# Autodesk Inventor assembly: Naped
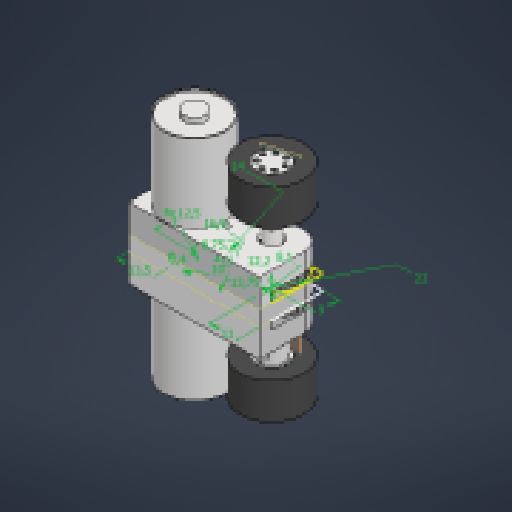
[picture p0: Inventor's stored thumbnail of the model, 512x512]
Saved by Autodesk Inventor 2023 (Build 270158000, 158)
## iProperties
Created: 2024-02-25
Part Number: Naped
Document SubType Name: Assembly
Designer: Michał
Author: Michał
## Documents named in this file (16)
- D:\Projekty\Roboilo\Ser\3D\3D\V2\Naped.iam
- D:\Projekty\Roboilo\Ser\3D\3D\V2\Naped\Przegroda.ipt
- D:\Projekty\Roboilo\Ser\3D\3D\V2\Naped\MocowaniePrzekladni.ipt
- D:\Projekty\Roboilo\Ser\3D\3D\PrzekladniaLewa\Design Accelerator\Przekładnie walcowe2.iam
- D:\Projekty\Roboilo\Ser\3D\3D\PrzekladniaLewa\Design Accelerator\Przekładnie walcowe3.iam
- D:\Projekty\Roboilo\Ser\3D\3D\PrzekladniaLewa\Design Accelerator\Przekładnie walcowe4.iam
- D:\Projekty\Roboilo\Ser\3D\3D\V2\Silnik.ipt
- D:\Projekty\Roboilo\Ser\3D\3D\V2\Naped\kolo.iam
- D:\Projekty\Roboilo\Ser\3D\3D\V2\Naped\Lozysko GFM-0608-06.ipt
- D:\Projekty\Roboilo\Ser\3D\3D\V2\Naped\MocowaniePrzekladni_MIR1.ipt
- D:\Projekty\Roboilo\Ser\3D\3D\V2\Silnik_MIR.ipt
- D:\Projekty\Roboilo\Ser\3D\3D\V2\Naped\kolo_MIR.iam
- D:\Projekty\Roboilo\Ser\3D\3D\PrzekladniaLewa\Design Accelerator\Przekładnie walcowe2_MIR.iam
- D:\Projekty\Roboilo\Ser\3D\3D\PrzekladniaLewa\Design Accelerator\Przekładnie walcowe3_MIR.iam
- D:\Projekty\Roboilo\Ser\3D\3D\PrzekladniaLewa\Design Accelerator\Przekładnie walcowe4_MIR.iam
- D:\Projekty\Roboilo\Ser\3D\3D\V2\Naped\Lozysko GFM-0608-06_MIR.ipt
## Components (15 placed, 13 different names)
1. Przegroda:1 — Flush:1, Flush:2, Mate:1, Mate:16, Flush:3, Flush:4
2. MocowaniePrzekladni:1 — Flush:1, Flush:2, Mate:1, Insert:1, Insert:2, Insert:3, Mate:3, Mate:4, Mate:5, Mate:6
3. Silnik:1 — Insert:1, Insert:2
4. kolo:1 [sub-assembly] — Mate:7, Mate:8
5. Przekładnie walcowe:1 [sub-assembly] — Insert:5, Mate:5, Mate:6
6. Przekładnie walcowe:2 [sub-assembly] — Insert:4, Insert:5, Mate:4
7. Przekładnie walcowe:3 [sub-assembly] — Insert:4, Mate:2, Mate:3, Mate:7, Mate:8
8. Lozysko GFM-0608-06:1 — Insert:3, Mate:2
9. MocowaniePrzekladni_MIR1:1 — Insert:6, Insert:7, Mate:9, Mate:10, Mate:11, Mate:14, Insert:10, Mate:16, Flush:3, Flush:4
10. Silnik_MIR:1 — Insert:6, Insert:7
11. kolo_MIR:1 [sub-assembly] — Mate:12, Mate:13
12. Przekładnie walcowe2_MIR:1 [sub-assembly] — Mate:9, Mate:10, Insert:8
13. Przekładnie walcowe3_MIR:1 [sub-assembly] — Mate:11, Insert:8, Insert:9
14. Przekładnie walcowe4_MIR:1 [sub-assembly] — Mate:12, Mate:13, Mate:14, Insert:9, Mate:15
15. Lozysko GFM-0608-06_MIR:1 — Mate:15, Insert:10
## Relationships (30: Mate 16, Insert 10, Flush 4)
- Flush:1: Przegroda:1 ↔ MocowaniePrzekladni:1
- Flush:2: Przegroda:1 ↔ MocowaniePrzekladni:1
- Mate:1: Przegroda:1 ↔ MocowaniePrzekladni:1
- Insert:1: MocowaniePrzekladni:1 ↔ Silnik:1
- Insert:2: MocowaniePrzekladni:1 ↔ Silnik:1
- Insert:3: MocowaniePrzekladni:1 ↔ Lozysko GFM-0608-06:1
- Insert:4: Przekładnie walcowe:2 ↔ Przekładnie walcowe:3
- Insert:5: Przekładnie walcowe:1 ↔ Przekładnie walcowe:2
- Mate:2: Przekładnie walcowe:3 ↔ Lozysko GFM-0608-06:1
- Mate:3: MocowaniePrzekladni:1 ↔ Przekładnie walcowe:3
- Mate:4: MocowaniePrzekladni:1 ↔ Przekładnie walcowe:2
- Mate:5: MocowaniePrzekladni:1 ↔ Przekładnie walcowe:1
- Mate:6 (0.1 mm): MocowaniePrzekladni:1 ↔ Przekładnie walcowe:1
- Mate:7: kolo:1 ↔ Przekładnie walcowe:3
- Mate:8: kolo:1 ↔ Przekładnie walcowe:3
- Insert:6: MocowaniePrzekladni_MIR1:1 ↔ Silnik_MIR:1
- Insert:7: MocowaniePrzekladni_MIR1:1 ↔ Silnik_MIR:1
- Mate:9 (0.1 mm): MocowaniePrzekladni_MIR1:1 ↔ Przekładnie walcowe2_MIR:1
- Mate:10: MocowaniePrzekladni_MIR1:1 ↔ Przekładnie walcowe2_MIR:1
- Mate:11: MocowaniePrzekladni_MIR1:1 ↔ Przekładnie walcowe3_MIR:1
- Insert:8: Przekładnie walcowe2_MIR:1 ↔ Przekładnie walcowe3_MIR:1
- Mate:12: kolo_MIR:1 ↔ Przekładnie walcowe4_MIR:1
- Mate:13: kolo_MIR:1 ↔ Przekładnie walcowe4_MIR:1
- Mate:14: MocowaniePrzekladni_MIR1:1 ↔ Przekładnie walcowe4_MIR:1
- Insert:9: Przekładnie walcowe3_MIR:1 ↔ Przekładnie walcowe4_MIR:1
- Mate:15: Przekładnie walcowe4_MIR:1 ↔ Lozysko GFM-0608-06_MIR:1
- Insert:10: MocowaniePrzekladni_MIR1:1 ↔ Lozysko GFM-0608-06_MIR:1
- Mate:16: Przegroda:1 ↔ MocowaniePrzekladni_MIR1:1
- Flush:3: Przegroda:1 ↔ MocowaniePrzekladni_MIR1:1
- Flush:4: Przegroda:1 ↔ MocowaniePrzekladni_MIR1:1
